# Autodesk Inventor assembly: motorAssembly01
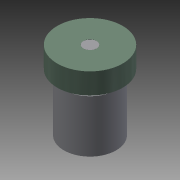
[picture p0: Inventor's stored thumbnail of the model, 180x180]
Saved by Autodesk Inventor 2013 (Build 170138000, 138)
## iProperties
Created: 2013-01-08
Part Number: motorAssembly01
Document SubType Name: Assembly
Designer: Nano
Author: Nano
## Documents named in this file (3)
- C:\Users\Nano\Documents\InventorByron\InventorMasterProject\gyroPhone01\motorAssembly01.iam
- C:\Users\Nano\Documents\InventorByron\InventorMasterProject\gyroPhone01\motorBodyAndShaft01.ipt
- C:\Users\Nano\Documents\InventorByron\InventorMasterProject\gyroPhone01\motorTire01.ipt
## Components (2 placed, 2 different names)
1. motorBodyAndShaft01:1 — Mate:1, Flush:1
2. motorTire01:1 — Mate:1, Flush:1
## Relationships (2: Mate 1, Flush 1)
- Mate:1: motorBodyAndShaft01:1 ↔ motorTire01:1
- Flush:1: motorBodyAndShaft01:1 ↔ motorTire01:1
